# Autodesk Inventor assembly: chassisstructure
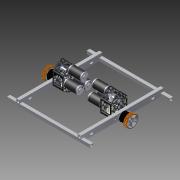
[picture p0: Inventor's stored thumbnail of the model, 180x180]
Saved by Autodesk Inventor 2014 SP1 (Build 180222100, 222)
## iProperties
Created: 2014-01-04
Part Number: chassisstructure
Document SubType Name: Assembly
Designer: Arpan
Mass: 17237.3 g
Surface Area: 13131.7 cm^2
Volume: 3885.03 cm^3
Density: 4.43684 g/cm^3
Author: Arpan
## Documents named in this file (5)
- C:\Users\Arpan\Documents\GitHub\2014buildCAD\chassisdrivetrain\chassis light\chassisstructure.iam
- C:\Users\Arpan\Documents\GitHub\2014buildCAD\chassisdrivetrain\chassis light\chassis front back rail.ipt
- C:\Users\Arpan\Documents\GitHub\2014buildCAD\chassisdrivetrain\chassis light\chassis side rail.ipt
- C:\Users\Arpan\Documents\GitHub\2014buildCAD\chassisdrivetrain\gearbot\3cimgearbox.iam
- C:\Users\Arpan\Documents\GitHub\2014buildCAD\chassisdrivetrain\chassis light\COTS items\center wheel assembly.iam
## Components (8 placed, 4 different names)
1. chassis front back rail:1 — Mate:5, Flush:4, Angle:1, Flush:5
2. chassis side rail:1 — Mate:3, Mate:4, Flush:2, Mate:5, Flush:4, Mate:6, Mate:7
3. chassis front back rail:2 — Flush:1, Mate:1, Mate:2, Mate:3, Mate:4, Flush:2, Flush:5
4. chassis side rail:2 — Flush:1, Mate:1, Mate:2, Mate:8, Mate:9
5. 3cimgearbox:1 [sub-assembly] — Mate:6, Mate:7, Angle:1, Angle:2, Flush:7, Mate:12, Mate:13
6. 3cimgearbox:2 [sub-assembly] — Mate:8, Mate:9, Angle:2, Flush:6, Mate:10, Mate:11
7. center wheel assembly:1 [sub-assembly] — Flush:6, Mate:10, Mate:11
8. center wheel assembly:2 [sub-assembly] — Flush:7, Mate:12, Mate:13
## Relationships (21: Mate 13, Flush 6, Angle 2)
- Flush:1 (-77.7494 mm): chassis front back rail:2 ↔ chassis side rail:2
- Mate:1: chassis front back rail:2 ↔ chassis side rail:2
- Mate:2: chassis front back rail:2 ↔ chassis side rail:2
- Mate:3: chassis side rail:1 ↔ chassis front back rail:2
- Mate:4: chassis side rail:1 ↔ chassis front back rail:2
- Flush:2 (-77.7494 mm): chassis side rail:1 ↔ chassis front back rail:2
- Mate:5: chassis front back rail:1 ↔ chassis side rail:1
- Flush:4: chassis front back rail:1 ↔ chassis side rail:1
- Mate:6: chassis side rail:1 ↔ 3cimgearbox:1
- Mate:7: chassis side rail:1 ↔ 3cimgearbox:1
- Angle:1 (0 deg): chassis front back rail:1 ↔ 3cimgearbox:1
- Mate:8: chassis side rail:2 ↔ 3cimgearbox:2
- Mate:9: chassis side rail:2 ↔ 3cimgearbox:2
- Angle:2 (0 deg): 3cimgearbox:1 ↔ 3cimgearbox:2
- Flush:5: chassis front back rail:1 ↔ chassis front back rail:2
- Flush:6: 3cimgearbox:2 ↔ center wheel assembly:1
- Mate:10: 3cimgearbox:2 ↔ center wheel assembly:1
- Mate:11: 3cimgearbox:2 ↔ center wheel assembly:1
- Flush:7: 3cimgearbox:1 ↔ center wheel assembly:2
- Mate:12: 3cimgearbox:1 ↔ center wheel assembly:2
- Mate:13: 3cimgearbox:1 ↔ center wheel assembly:2
